# Autodesk Inventor assembly: Assembly1
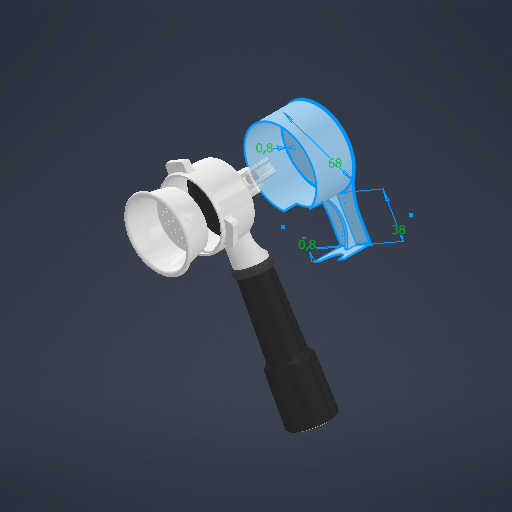
[picture p0: Inventor's stored thumbnail of the model, 512x512]
Saved by Autodesk Inventor 2026 (Build 300175000, 175)
## iProperties
Created: 2025-04-15
Part Number: Assembly1
Document SubType Name: Assembly
Designer: Paul Juschitz
Author: Paul Juschitz
## Documents named in this file (3)
- C:\Users\Paul Juschitz\Documents\private\m5_GBW_mod\M5_GBW_mod\CAD\Assembly1.iam
- C:\Users\Paul Juschitz\Documents\private\m5_GBW_mod\M5_GBW_mod\CAD\my_portafilter_holder.ipt
- C:\Users\Paul Juschitz\Documents\private\m5_GBW_mod\M5_GBW_mod\CAD\downloads\portafilter\BES870XL Portafilter\BES870XL Portafilter\BES870XL Portafilter.iam
## Components (2 placed, 2 different names)
1. my_portafilter_holder:1 — Angle:1, Angle:2, Cylindrical:1
2. BES870XL Portafilter:1 [sub-assembly] — Angle:1, Angle:2, Cylindrical:1
## Relationships (3: Angle 2, CylindricalJoint 1)
- Angle:1 (180 deg): my_portafilter_holder:1 ↔ BES870XL Portafilter:1
- Angle:2 (180 deg): my_portafilter_holder:1 ↔ BES870XL Portafilter:1
- Cylindrical:1: my_portafilter_holder:1 ↔ BES870XL Portafilter:1
